# Autodesk Inventor assembly: attachementToTripodWithInserts
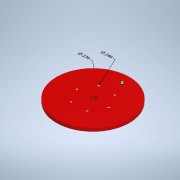
[picture p0: Inventor's stored thumbnail of the model, 180x180]
Saved by Autodesk Inventor 2022.2 (Build 262287010, 287A)
## iProperties
Created: 2021-03-14
Part Number: attachementToTripodWithInserts
Document SubType Name: Assembly
Designer: robst
Author: robst
## Documents named in this file (4)
- C:\git\CAD-Development\robSteele\ShapeWays\TelescopeProjects\TelescopeMountNov2020\attachementToTripodWithInserts.iam
- C:\git\CAD-Development\robSteele\ShapeWays\TelescopeProjects\TelescopeMountNov2020\attachementToTripod.ipt
- C:\git\CAD-Development\robSteele\ShapeWays\TelescopeProjects\TelescopeMountNov2020\10-32x0_310_BRASS HEAT-SET INSERT FOR PLASTIC.ipt
- C:\git\CAD-Development\robSteele\ShapeWays\TelescopeProjects\TelescopeMountNov2020\90592A024_STEEL HEX NUT.ipt
## Components (8 placed, 3 different names)
1. attachementToTripod:1 — Mate:1, Insert:1, Mate:2, Mate:3
2. 90592A024_STEEL HEX NUT:1 — Mate:2, Mate:3
3. 10-32x0_310_BRASS HEAT-SET INSERT FOR PLASTIC:1 — Insert:1
4. 10-32x0_310_BRASS HEAT-SET INSERT FOR PLASTIC:2
5. 10-32x0_310_BRASS HEAT-SET INSERT FOR PLASTIC:3
6. 10-32x0_310_BRASS HEAT-SET INSERT FOR PLASTIC:4
7. 10-32x0_310_BRASS HEAT-SET INSERT FOR PLASTIC:5
8. 10-32x0_310_BRASS HEAT-SET INSERT FOR PLASTIC:6
## Component patterns: (6 elements, first: 10-32x0_310_BRASS HEAT-SET INSERT FOR PLASTIC:1)
## Relationships (4: Mate 3, Insert 1)
- Mate:1: attachementToTripod:1
- Insert:1: attachementToTripod:1 ↔ 10-32x0_310_BRASS HEAT-SET INSERT FOR PLASTIC:1
- Mate:2: attachementToTripod:1 ↔ 90592A024_STEEL HEX NUT:1
- Mate:3: attachementToTripod:1 ↔ 90592A024_STEEL HEX NUT:1
